# Autodesk Inventor assembly: Wózek_inwalidzki
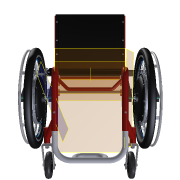
[picture p0: Inventor's stored thumbnail of the model, 180x180]
Saved by Autodesk Inventor 2015 (Build 190159000, 159)
## iProperties
Created: 2016-01-12
Part Number: Wózek_inwalidzki
Document SubType Name: Assembly
Designer: graaapsik
Author: graaapsik
## Documents named in this file (29)
- C:\Users\EriveltonDell\Documents\Centro Universitário da FEI\Wheelchair\CADEIRA DE RODAS - DESENHO\GITHUB\Montagem com Garfo Retangular.iam
- C:\Users\EriveltonDell\Documents\Centro Universitário da FEI\Wheelchair\CADEIRA DE RODAS - DESENHO\GITHUB\Hamulec.iam
- C:\Users\EriveltonDell\Documents\Centro Universitário da FEI\Wheelchair\CADEIRA DE RODAS - DESENHO\GITHUB\Koło_przednie.iam
- C:\Users\EriveltonDell\Documents\Centro Universitário da FEI\Wheelchair\CADEIRA DE RODAS - DESENHO\GITHUB\Rama_wozka.iam
- C:\Users\EriveltonDell\Documents\Centro Universitário da FEI\Wheelchair\CADEIRA DE RODAS - DESENHO\GITHUB\Tapicerka_oparcia.iam
- C:\Users\EriveltonDell\Documents\Centro Universitário da FEI\Wheelchair\CADEIRA DE RODAS - DESENHO\GITHUB\Tapicerka_siedziska.iam
- C:\Users\EriveltonDell\Documents\Centro Universitário da FEI\Wheelchair\CADEIRA DE RODAS - DESENHO\GITHUB\Ciąg.iam
- C:\Users\EriveltonDell\Documents\Centro Universitário da FEI\Wheelchair\CADEIRA DE RODAS - DESENHO\GITHUB\Widelec.iam
- C:\Users\EriveltonDell\Documents\Centro Universitário da FEI\Wheelchair\CADEIRA DE RODAS - DESENHO\GITHUB\Zaślepka_do_widelca.ipt
- C:\Users\EriveltonDell\Documents\Centro Universitário da FEI\Wheelchair\CADEIRA DE RODAS - DESENHO\GITHUB\Podnóżek.iam
- C:\Users\EriveltonDell\Documents\Centro Universitário da FEI\Wheelchair\CADEIRA DE RODAS - DESENHO\GITHUB\Zaślepka_do_rur_fi32.ipt
- C:\Users\EriveltonDell\Documents\Centro Universitário da FEI\Wheelchair\CADEIRA DE RODAS - DESENHO\GITHUB\suporte-rodas-esq.ipt
- C:\Users\EriveltonDell\Documents\Centro Universitário da FEI\Wheelchair\CADEIRA DE RODAS - DESENHO\GITHUB\suporte-rodas.ipt
- C:\Users\EriveltonDell\Documents\Centro Universitário da FEI\Wheelchair\CADEIRA DE RODAS - DESENHO\GITHUB\suporte-eixo.ipt
- C:\Users\EriveltonDell\Documents\Centro Universitário da FEI\Wheelchair\CADEIRA DE RODAS - DESENHO\GITHUB\Barra-garfo.ipt
- C:\Users\EriveltonDell\Documents\Centro Universitário da FEI\Wheelchair\CADEIRA DE RODAS - DESENHO\GITHUB\suporte-eixo - 2.ipt
- C:\Users\EriveltonDell\Documents\Centro Universitário da FEI\Wheelchair\CADEIRA DE RODAS - DESENHO\GITHUB\ISO 4032 - M12ISO.ipt
- C:\Users\EriveltonDell\Documents\Centro Universitário da FEI\Wheelchair\CADEIRA DE RODAS - DESENHO\GITHUB\GARFO - Copy.ipt
- C:\Users\EriveltonDell\Documents\Centro Universitário da FEI\Wheelchair\CADEIRA DE RODAS - DESENHO\GITHUB\edge.ipt
- C:\Users\EriveltonDell\Documents\Centro Universitário da FEI\Wheelchair\CADEIRA DE RODAS - DESENHO\GITHUB\motorEaro.iam
- C:\Users\EriveltonDell\Documents\Centro Universitário da FEI\Wheelchair\CADEIRA DE RODAS - DESENHO\GITHUB\Imported Components\Hub_Motor_MagicPie2_ASM\Hub_Motor_MagicPie2_ASM.iam
- C:\Users\EriveltonDell\Documents\Centro Universitário da FEI\Wheelchair\CADEIRA DE RODAS - DESENHO\GITHUB\Barra-superior.ipt
- C:\Users\EriveltonDell\Documents\Centro Universitário da FEI\Wheelchair\CADEIRA DE RODAS - DESENHO\GITHUB\pino.ipt
- C:\Users\EriveltonDell\Documents\Centro Universitário da FEI\Wheelchair\CADEIRA DE RODAS - DESENHO\GITHUB\Chapa Pino.ipt
- C:\Users\EriveltonDell\Documents\Centro Universitário da FEI\Wheelchair\CADEIRA DE RODAS - DESENHO\GITHUB\suporte-barra - tampa.ipt
- C:\Users\EriveltonDell\Documents\Centro Universitário da FEI\Wheelchair\CADEIRA DE RODAS - DESENHO\GITHUB\Abraca estrutura.ipt
- C:\Users\EriveltonDell\Documents\Centro Universitário da FEI\Wheelchair\CADEIRA DE RODAS - DESENHO\GITHUB\Abraca estrutura - comp.ipt
- C:\Users\EriveltonDell\Documents\Centro Universitário da FEI\Wheelchair\CADEIRA DE RODAS - DESENHO\GITHUB\Abraca estrutura - 20.ipt
- C:\Users\EriveltonDell\Documents\Centro Universitário da FEI\Wheelchair\CADEIRA DE RODAS - DESENHO\GITHUB\Luva new.ipt
## Components (52 placed, 28 different names)
1. Rama_wozka:1 [sub-assembly] — Zestawiający:7, Zestawiający:8, Zestawiający:9, Zestawiający:10, Zestawiający:11, Zestawiający:12, Równoległy:1, Zestawiający:15, Symetria:1, Równoległy:2, Zestawiający:20, Zestawiający:22, Zestawiający:27, Zestawiający:29, Zestawiający:36, Zestawiający:37, Równoległy:3, Zestawiający:38, Zestawiający:39, Zestawiający:40, Zestawiający:41, Zestawiający:42, Zestawiający:43, Zestawiający:44, Zestawiający:45, Angle:9, Insert:13, Insert:14, Insert:30, Insert:31, Mate:143, Mate:144
2. Ciąg:1 [sub-assembly]
3. Ciąg:2 [sub-assembly]
4. Widelec:1 [sub-assembly] — Zestawiający:9, Zestawiający:11, Wstaw:3
5. Widelec:2 [sub-assembly] — Zestawiający:10, Zestawiający:12, Zestawiający:13, Zestawiający:14, Symetria:1
6. Koło_przednie:1 [sub-assembly] — Wstaw:3
7. Koło_przednie:2 [sub-assembly] — Zestawiający:13, Zestawiający:14
8. Hamulec:1 [sub-assembly] — Zestawiający:38, Zestawiający:39, Angle:9
9. Tapicerka_oparcia:1 [sub-assembly] — Równoległy:1, Zestawiający:16
10. Tapicerka_siedziska:1 [sub-assembly] — Zestawiający:15, Zestawiający:16, Angle:10, Angle:11
11. Zaślepka_do_widelca:1 — Zestawiający:8, Zestawiający:45
12. Zaślepka_do_widelca:2 — Zestawiający:7, Zestawiający:44
13. Podnóżek:1 [sub-assembly] — Zestawiający:36, Zestawiający:37, Równoległy:3
14. Zaślepka_do_rur_fi32:1 — Zestawiający:22, Zestawiający:42
15. Zaślepka_do_rur_fi32:2 — Zestawiający:27, Zestawiający:40
16. Zaślepka_do_rur_fi32:3 — Zestawiający:20, Zestawiający:43
17. Zaślepka_do_rur_fi32:5 — Zestawiający:29, Zestawiający:41
18. suporte-rodas-esq:1 — Insert:14, Angle:10, Mate:55, Tangent:19, Tangent:20
19. suporte-rodas:1 — Insert:13, Angle:11, Mate:62, Tangent:21, Tangent:22
20. suporte-eixo:2 — Mate:55, Tangent:19, Tangent:20, Insert:33
21. suporte-eixo - 2:1 — Mate:62, Tangent:21, Tangent:22, Mate:118
22. Zaślepka_do_rur_fi32:6 — Insert:30
23. Zaślepka_do_rur_fi32:7 — Insert:31
24. ISO 4032 M12:1 — Mate:151, Mate:152
25. GARFO - Copy:1 — Flush:5, Flush:6, Mate:94, Mate:95, Mate:96, Mate:97, Mate:98, Mate:113, Mate:114, Flush:10, Mate:122, Mate:129, Mate:152, Flush:34, Mate:156, Mate:162, Mate:163, Mate:164, Mate:172
26. GARFO - Copy:2 — Flush:5, Mate:99, Mate:100, Mate:101, Mate:102, Flush:7, Flush:8, Mate:112, Mate:115, Mate:116, Flush:9, Mate:120, Mate:124, Mate:154, Flush:33, Mate:157, Mate:159, Mate:160, Mate:161, Mate:170, Mate:174
27. edge:1 — Flush:6, Mate:94, Mate:95
28. edge:2 — Mate:96, Mate:97, Mate:98
29. edge:3 — Mate:101, Mate:102, Flush:7
30. edge:4 — Mate:99, Mate:100, Flush:8
31. Ciąg:3 [sub-assembly]
32. motorEaro:1 [sub-assembly] — Mate:112
33. Hub_Motor_MagicPie2_ASM:2 [sub-assembly] — Mate:113, Mate:114, Mate:117, Mate:151, Mate:171
34. Hub_Motor_MagicPie2_ASM:3 [sub-assembly] — Mate:115, Mate:116, Mate:117, Mate:153, Mate:173
35. Barra-superior:1 — Mate:118, Mate:121, Mate:123, Mate:156, Insert:33, Mate:157
36. pino:1 — Flush:9, Mate:120, Mate:121, Mate:125
37. pino:2 — Flush:10, Mate:122, Mate:123, Mate:130
38. Chapa Pino:1 — Mate:124, Mate:125, Flush:33
39. Chapa Pino:2 — Mate:129, Mate:130, Flush:34
40. Abraca estrutura - comp:1 — Mate:158, Flush:37, Mate:169, Flush:44, Flush:45, Flush:46
41. Abraca estrutura - 20:1 — Mate:143, Flush:35, Flush:36, Mate:158, Flush:37, Flush:44
42. Abraca estrutura - 20:2 — Mate:144, Flush:35, Flush:36
43. ISO 4032 M12:2 — Mate:153, Mate:154
44. suporte-barra - tampa:2 — Mate:164, Flush:40, Flush:41
45. suporte-barra - tampa:3 — Mate:161, Flush:38, Flush:39
46. Abraca estrutura:1 — Mate:167, Flush:42, Flush:43
47. Abraca estrutura:2 — Mate:168, Flush:42, Flush:43, Mate:169, Flush:45, Flush:46, Mate:176
48. Barra-garfo:1 — Mate:167, Mate:168, Mate:175, Insert:34
49. Luva new:1 — Mate:159, Mate:160, Flush:38, Flush:39, Mate:170, Insert:34, Mate:176
50. Luva new:2 — Mate:162, Mate:163, Flush:40, Flush:41, Mate:175
51. ISO 4032 M12:3 — Mate:171, Mate:172
52. ISO 4032 M12:4 — Mate:173, Mate:174
## Relationships (113: Mate 75, Flush 23, Insert 7, Tangent 4, Angle 3, Symmetry 1)
- Zestawiający:7 [Mate]: Rama_wozka:1 ↔ Zaślepka_do_widelca:2
- Zestawiający:8 [Mate]: Rama_wozka:1 ↔ Zaślepka_do_widelca:1
- Zestawiający:9 [Mate]: Rama_wozka:1 ↔ Widelec:1
- Zestawiający:10 [Mate]: Rama_wozka:1 ↔ Widelec:2
- Zestawiający:11 [Mate]: Rama_wozka:1 ↔ Widelec:1
- Zestawiający:12 [Mate]: Rama_wozka:1 ↔ Widelec:2
- Zestawiający:13 [Mate]: Widelec:2 ↔ Koło_przednie:2
- Zestawiający:14 [Mate]: Widelec:2 ↔ Koło_przednie:2
- Równoległy:1 [Flush] (-16 mm): Rama_wozka:1 ↔ Tapicerka_oparcia:1
- Zestawiający:15 [Mate] (16 mm): Rama_wozka:1 ↔ Tapicerka_siedziska:1
- Zestawiający:16 [Mate] (0.25 mm): Tapicerka_oparcia:1 ↔ Tapicerka_siedziska:1
- Symetria:1 [Symmetry]: Rama_wozka:1 ↔ Widelec:2
- Równoległy:2 [Flush]: Rama_wozka:1
- Zestawiający:20 [Mate]: Rama_wozka:1 ↔ Zaślepka_do_rur_fi32:3
- Zestawiający:22 [Mate]: Rama_wozka:1 ↔ Zaślepka_do_rur_fi32:1
- Zestawiający:27 [Mate]: Rama_wozka:1 ↔ Zaślepka_do_rur_fi32:2
- Zestawiający:29 [Mate]: Rama_wozka:1 ↔ Zaślepka_do_rur_fi32:5
- Wstaw:3 [Insert]: Widelec:1 ↔ Koło_przednie:1
- Zestawiający:36 [Mate]: Rama_wozka:1 ↔ Podnóżek:1
- Zestawiający:37 [Mate]: Rama_wozka:1 ↔ Podnóżek:1
- Równoległy:3 [Flush] (150 mm): Rama_wozka:1 ↔ Podnóżek:1
- Zestawiający:38 [Mate]: Rama_wozka:1 ↔ Hamulec:1
- Zestawiający:39 [Mate] (40 mm): Rama_wozka:1 ↔ Hamulec:1
- Zestawiający:40 [Mate]: Rama_wozka:1 ↔ Zaślepka_do_rur_fi32:2
- Zestawiający:41 [Mate]: Rama_wozka:1 ↔ Zaślepka_do_rur_fi32:5
- Zestawiający:42 [Mate]: Rama_wozka:1 ↔ Zaślepka_do_rur_fi32:1
- Zestawiający:43 [Mate]: Rama_wozka:1 ↔ Zaślepka_do_rur_fi32:3
- Zestawiający:44 [Mate]: Rama_wozka:1 ↔ Zaślepka_do_widelca:2
- Zestawiający:45 [Mate]: Rama_wozka:1 ↔ Zaślepka_do_widelca:1
- Angle:9 (0 deg): Rama_wozka:1 ↔ Hamulec:1
- Insert:13 (150 mm): Rama_wozka:1 ↔ suporte-rodas:1
- Insert:14 (150 mm): Rama_wozka:1 ↔ suporte-rodas-esq:1
- Angle:10 (90 deg): Tapicerka_siedziska:1 ↔ suporte-rodas-esq:1
- Angle:11 (90 deg): Tapicerka_siedziska:1 ↔ suporte-rodas:1
- Mate:55: suporte-rodas-esq:1 ↔ suporte-eixo:2
- Tangent:19: suporte-rodas-esq:1 ↔ suporte-eixo:2
- Tangent:20: suporte-rodas-esq:1 ↔ suporte-eixo:2
- Mate:62: suporte-rodas:1 ↔ suporte-eixo - 2:1
- Tangent:21: suporte-rodas:1 ↔ suporte-eixo - 2:1
- Tangent:22: suporte-rodas:1 ↔ suporte-eixo - 2:1
- Insert:30 (-8 mm): Rama_wozka:1 ↔ Zaślepka_do_rur_fi32:6
- Insert:31 (-8 mm): Rama_wozka:1 ↔ Zaślepka_do_rur_fi32:7
- Flush:5: GARFO - Copy:1 ↔ GARFO - Copy:2
- Flush:6: GARFO - Copy:1 ↔ edge:1
- Mate:94: GARFO - Copy:1 ↔ edge:1
- Mate:95: GARFO - Copy:1 ↔ edge:1
- Mate:96: GARFO - Copy:1 ↔ edge:2
- Mate:97: GARFO - Copy:1 ↔ edge:2
- Mate:98: GARFO - Copy:1 ↔ edge:2
- Mate:99: GARFO - Copy:2 ↔ edge:4
- Mate:100: GARFO - Copy:2 ↔ edge:4
- Mate:101: GARFO - Copy:2 ↔ edge:3
- Mate:102: GARFO - Copy:2 ↔ edge:3
- Flush:7: GARFO - Copy:2 ↔ edge:3
- Flush:8: GARFO - Copy:2 ↔ edge:4
- Mate:112: GARFO - Copy:2 ↔ motorEaro:1
- Mate:113: GARFO - Copy:1 ↔ Hub_Motor_MagicPie2_ASM:2
- Mate:114 (8 mm): GARFO - Copy:1 ↔ Hub_Motor_MagicPie2_ASM:2
- Mate:115: GARFO - Copy:2 ↔ Hub_Motor_MagicPie2_ASM:3
- Mate:116 (8 mm): GARFO - Copy:2 ↔ Hub_Motor_MagicPie2_ASM:3
- Mate:117: Hub_Motor_MagicPie2_ASM:2 ↔ Hub_Motor_MagicPie2_ASM:3
- Mate:118: suporte-eixo - 2:1 ↔ Barra-superior:1
- Flush:9: GARFO - Copy:2 ↔ pino:1
- Mate:120: GARFO - Copy:2 ↔ pino:1
- Mate:121: Barra-superior:1 ↔ pino:1
- Flush:10: GARFO - Copy:1 ↔ pino:2
- Mate:122: GARFO - Copy:1 ↔ pino:2
- Mate:123: Barra-superior:1 ↔ pino:2
- Mate:124: GARFO - Copy:2 ↔ Chapa Pino:1
- Mate:125: pino:1 ↔ Chapa Pino:1
- Mate:129: GARFO - Copy:1 ↔ Chapa Pino:2
- Mate:130: pino:2 ↔ Chapa Pino:2
- Mate:143: Rama_wozka:1 ↔ Abraca estrutura - 20:1
- Mate:144: Rama_wozka:1 ↔ Abraca estrutura - 20:2
- Mate:151: ISO 4032 M12:1 ↔ Hub_Motor_MagicPie2_ASM:2
- Mate:152: ISO 4032 M12:1 ↔ GARFO - Copy:1
- Mate:153: Hub_Motor_MagicPie2_ASM:3 ↔ ISO 4032 M12:2
- Mate:154: GARFO - Copy:2 ↔ ISO 4032 M12:2
- Flush:33: GARFO - Copy:2 ↔ Chapa Pino:1
- Flush:34: GARFO - Copy:1 ↔ Chapa Pino:2
- Mate:156: GARFO - Copy:1 ↔ Barra-superior:1
- Insert:33 (-18 mm): suporte-eixo:2 ↔ Barra-superior:1
- Mate:157: GARFO - Copy:2 ↔ Barra-superior:1
- Flush:35: Abraca estrutura - 20:1 ↔ Abraca estrutura - 20:2
- Flush:36: Abraca estrutura - 20:1 ↔ Abraca estrutura - 20:2
- Mate:158: Abraca estrutura - comp:1 ↔ Abraca estrutura - 20:1
- Flush:37: Abraca estrutura - comp:1 ↔ Abraca estrutura - 20:1
- Mate:159 (0.25 mm): GARFO - Copy:2 ↔ Luva new:1
- Mate:160: GARFO - Copy:2 ↔ Luva new:1
- Mate:161: GARFO - Copy:2 ↔ suporte-barra - tampa:3
- Flush:38: suporte-barra - tampa:3 ↔ Luva new:1
- Flush:39: suporte-barra - tampa:3 ↔ Luva new:1
- Mate:162 (0.25 mm): GARFO - Copy:1 ↔ Luva new:2
- Mate:163: GARFO - Copy:1 ↔ Luva new:2
- Mate:164: GARFO - Copy:1 ↔ suporte-barra - tampa:2
- Flush:40: suporte-barra - tampa:2 ↔ Luva new:2
- Flush:41: suporte-barra - tampa:2 ↔ Luva new:2
- Mate:167: Abraca estrutura:1 ↔ Barra-garfo:1
- Mate:168: Abraca estrutura:2 ↔ Barra-garfo:1
- Flush:42: Abraca estrutura:1 ↔ Abraca estrutura:2
- Flush:43: Abraca estrutura:1 ↔ Abraca estrutura:2
- Mate:169: Abraca estrutura - comp:1 ↔ Abraca estrutura:2
- Flush:44 (-15 mm): Abraca estrutura - comp:1 ↔ Abraca estrutura - 20:1
- Mate:170 (10 mm): GARFO - Copy:2 ↔ Luva new:1
- Flush:45: Abraca estrutura - comp:1 ↔ Abraca estrutura:2
- Flush:46: Abraca estrutura - comp:1 ↔ Abraca estrutura:2
- Mate:171: Hub_Motor_MagicPie2_ASM:2 ↔ ISO 4032 M12:3
- Mate:172: GARFO - Copy:1 ↔ ISO 4032 M12:3
- Mate:173: Hub_Motor_MagicPie2_ASM:3 ↔ ISO 4032 M12:4
- Mate:174: GARFO - Copy:2 ↔ ISO 4032 M12:4
- Mate:175: Barra-garfo:1 ↔ Luva new:2
- Insert:34: Barra-garfo:1 ↔ Luva new:1
- Mate:176 (180 mm): Abraca estrutura:2 ↔ Luva new:1
## Named parameters: sa_0 = 1.6e-12, sa_1 = -6.84e-11, sa_2 = -70000
note: some values were not read from the file. Shown as the stored number, unit unknown: "sa_0", "sa_1", "sa_2".
